# Autodesk Inventor assembly: Assembly2
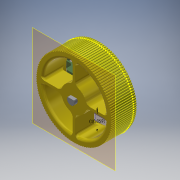
[picture p0: Inventor's stored thumbnail of the model, 180x180]
Saved by Autodesk Inventor 2019 (Build 230136000, 136)
## iProperties
Created: 2019-09-12
Part Number: Assembly2
Document SubType Name: Assembly
Designer: assman
Author: assman
## Documents named in this file (4)
- D:\Inventor\Projects\ArduSpinner\Assembly2.iam
- D:\Inventor\Projects\ArduSpinner\wheel.ipt
- D:\Inventor\Projects\ArduSpinner\encoder.ipt
- D:\Inventor\Projects\chassis2.ipt
## Components (3 placed, 3 different names)
1. wheel:1 — Rotational:1
2. encoder:1 — Flush:1, Rotational:1, Flush:2
3. chassis2:1 — Flush:3, Flush:4
## Relationships (5: Flush 4, RevoluteJoint 1)
- Flush:1: encoder:1
- Rotational:1 [RevoluteJoint] (-5 mm): wheel:1 ↔ encoder:1
- Flush:2: encoder:1
- Flush:3: chassis2:1
- Flush:4: chassis2:1
